# Autodesk Inventor assembly: Assembly1
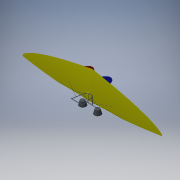
[picture p0: Inventor's stored thumbnail of the model, 180x180]
Saved by Autodesk Inventor 2016 (Build 200138000, 138)
## iProperties
Created: 2016-05-15
Part Number: Assembly1
Document SubType Name: Assembly
Designer: Mauricio
Author: Mauricio
## Documents named in this file (4)
- C:\Users\Mauricio\Downloads\spaceapps\Assembly1.iam
- C:\Users\Mauricio\Downloads\spaceapps\Part1.ipt
- C:\Users\Mauricio\Downloads\spaceapps\Part2.ipt
- C:\Users\Mauricio\Downloads\spaceapps\Part4.ipt
## Components (4 placed, 3 different names)
1. Part1:1 — Rotational:1, Rotational:2, Rotational:3
2. Part2:1 — Rotational:2
3. Part2:2 — Rotational:1
4. Part4:1 — Rotational:3
## Relationships (3: RevoluteJoint 3)
- Rotational:1 [RevoluteJoint]: Part1:1 ↔ Part2:2
- Rotational:2 [RevoluteJoint]: Part1:1 ↔ Part2:1
- Rotational:3 [RevoluteJoint] (-200 mm): Part1:1 ↔ Part4:1
